# Autodesk Inventor assembly: BBM Staging Plate Assembly
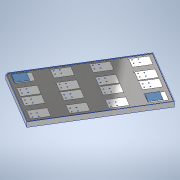
[picture p0: Inventor's stored thumbnail of the model, 180x180]
Saved by Autodesk Inventor 2022 (Build 260153000, 153)
## iProperties
Created: 2021-01-11
Part Number: BBM Staging Plate Assembly
Document SubType Name: Assembly
Designer: caleb
Author: caleb
## Documents named in this file (4)
- C:\Users\Caleb\Desktop\nebraska-silicon-lab\Hardware\ETL\Module Assembly\BBM Staging Plate - V2\BBM Staging Plate Assembly - V2.iam
- C:\Users\Caleb\Desktop\nebraska-silicon-lab\Hardware\ETL\Module Assembly\BBM Staging Plate - V2\BBM Staging Plate - V2.ipt
- C:\Users\Caleb\Desktop\nebraska-silicon-lab\Hardware\ETL\Module Assembly\BBM Staging Plate - V2\BBM Staging Plate Stencil - V2.ipt
- C:\Users\Caleb\Desktop\nebraska-silicon-lab\Hardware\ETL\Module Assembly\BBM Staging Plate - V2\F10112319--_1-MODULE_ CMS2 ETL_ PIXEL SENSOR READOUT CHIP.ipt
## Components (4 placed, 3 different names)
1. BBM Staging Plate - V2:1 — Mate:8, Mate:11
2. BBM Staging Plate Stencil - V2:1 — Mate:6, Mate:7, Mate:9, Mate:10, Mate:11
3. F10112319--_1-MODULE_ CMS2 ETL_ PIXEL SENSOR READOUT CHIP:1 — Mate:6, Mate:7
4. F10112319--_1-MODULE_ CMS2 ETL_ PIXEL SENSOR READOUT CHIP:2 — Mate:8, Mate:9, Mate:10
## Relationships (6: Mate 6)
- Mate:6: BBM Staging Plate Stencil - V2:1 ↔ F10112319--_1-MODULE_ CMS2 ETL_ PIXEL SENSOR READOUT CHIP:1
- Mate:7: BBM Staging Plate Stencil - V2:1 ↔ F10112319--_1-MODULE_ CMS2 ETL_ PIXEL SENSOR READOUT CHIP:1
- Mate:8: BBM Staging Plate - V2:1 ↔ F10112319--_1-MODULE_ CMS2 ETL_ PIXEL SENSOR READOUT CHIP:2
- Mate:9: BBM Staging Plate Stencil - V2:1 ↔ F10112319--_1-MODULE_ CMS2 ETL_ PIXEL SENSOR READOUT CHIP:2
- Mate:10: BBM Staging Plate Stencil - V2:1 ↔ F10112319--_1-MODULE_ CMS2 ETL_ PIXEL SENSOR READOUT CHIP:2
- Mate:11: BBM Staging Plate - V2:1 ↔ BBM Staging Plate Stencil - V2:1
